# Autodesk Inventor assembly: Подъёмник
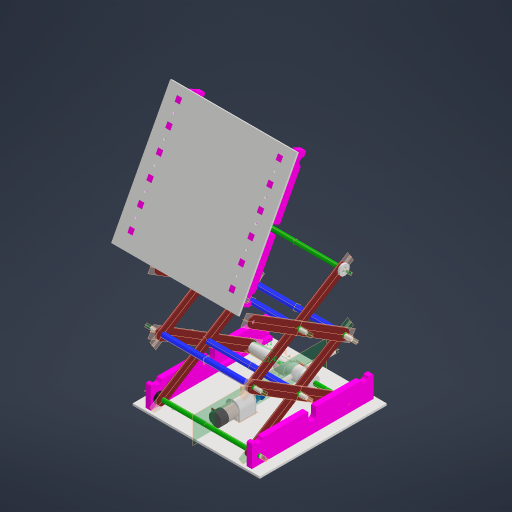
[picture p0: Inventor's stored thumbnail of the model, 512x512]
Saved by Autodesk Inventor 2023.2 (Build 272271030, 271C)
## iProperties
Created: 2025-03-18
Part Number: Подъёмник
Document SubType Name: Assembly
Designer: Коноваленко
Author: Коноваленко
## Documents named in this file (18)
- D:\!Rover\Rover\Rover_construction\Подъёмник.iam
- D:\!Rover\Rover\Rover_construction\Рельс платформы подъёмника.ipt
- D:\!Rover\Rover\Rover_construction\Рычаг платформы подъёмника.ipt
- D:\!Rover\Rover\Rover_construction\Основание подъёмника.ipt
- D:\!Rover\Rover\Rover_construction\Трубка.ipt
- D:\!Rover\Rover\Rover_construction\Рельс платформы подъёмника_MIR.ipt
- D:\!Rover\Rover\Rover_construction\Бабышка.ipt
- D:\!Rover\Rover\Rover_construction\Рельс платформы подъёмника_MIR1.ipt
- D:\!Rover\Rover\Rover_construction\Трубка основания.ipt
- D:\!Rover\Rover\Rover_construction\Подшипник.ipt
- D:\!Rover\Rover\Rover_construction\шпилька 6мм.ipt
- D:\!Rover\Rover\Rover_construction\Уголок крепления мотора.ipt
- D:\!Rover\Rover\Rover_construction\25d-metal-gearmotor-20.4-encoder.ipt
- D:\!Rover\Rover\Rover_construction\ftulka.ipt
- D:\!Rover\Rover\Rover_construction\Трапециевидный винт.ipt
- D:\!Rover\Rover\Rover_construction\Крепление ходовой гайки.ipt
- D:\!Rover\Rover\Rover_construction\THSL-300-8D õîäîâàÿ ãàéêà.ipt
- D:\!Rover\Rover\Rover_construction\Стакан для крепления ходовой гайки.ipt
## Components (60 placed, 17 different names)
1. Рельс платформы подъёмника:1 — Совмещение:63, Совмещение:64
2. Платформа подъёмника:1 — Совмещение:9, Заподлицо:8, Заподлицо:9, Заподлицо:12, Заподлицо:13, Совмещение:16, Совмещение:17, Заподлицо:14, Заподлицо:15, Совмещение:44, Заподлицо:21, Заподлицо:22
3. Рельс платформы подъёмника:4 — Совмещение:9, Заподлицо:8, Заподлицо:9, С поворотом:32, Ползун:3, Симметрия:1
4. Трубка:1 — С поворотом:82
5. Трубка:2 — С поворотом:79
6. Рельс платформы подъёмника_MIR:1 — Совмещение:65, Совмещение:66, С поворотом:86, Совмещение:81
7. Рельс платформы подъёмника_MIR1:1 — Заподлицо:12, Заподлицо:13, Совмещение:16, С поворотом:33, Ползун:4, Симметрия:1
8. Бабышка:9 — С поворотом:33, С поворотом:34
9. Бабышка:10 — С поворотом:32, С поворотом:37
10. Трубка основания:1 — С поворотом:75
11. Трубка основания:2
12. Подшипник:1 — С поворотом:70
13. Подшипник:2
14. Подшипник:3 — Ползун:3, Цилиндрический:4
15. Подшипник:4 — Ползун:4, Цилиндрический:6
16. Трубка основания:3 — С поворотом:77
17. Трубка:3 — С поворотом:72, С поворотом:77
18. Трубка:5 — С поворотом:74
19. Трубка основания:4 — С поворотом:83
20. Трубка основания:5 — С поворотом:66, С поворотом:69
21. Трубка:6 — С поворотом:54
22. Трубка:7 — С поворотом:73
23. Трубка основания:6 — Совмещение:28, Совмещение:29
24. Трубка основания:7 — С поворотом:85
25. Трубка:8 — С поворотом:53, Совмещение:28
26. Трубка:9 — Цилиндрический:2, С поворотом:66
27. шпилька 6мм:3 — С поворотом:69, С поворотом:70
28. Трубка:10 — С поворотом:84, С поворотом:85, С поворотом:86
29. Трубка основания:8 — С поворотом:80
30. Бабышка:11 — С поворотом:60
31. Бабышка:12 — С поворотом:61
32. шпилька 6мм:4 — С поворотом:71, С поворотом:72
33. шпилька 6мм:5 — С поворотом:73
34. шпилька 6мм:6 — С поворотом:74, С поворотом:75, С поворотом:76
35. шпилька 6мм:7 — С поворотом:81, С поворотом:82, С поворотом:83
36. шпилька 6мм:8 — С поворотом:84
37. шпилька 6мм:9 — С поворотом:78, С поворотом:79, С поворотом:80
38. Уголок крепления мотора:1 — Совмещение:44, Заподлицо:21, Совмещение:45, Совмещение:46, Совмещение:47, Совмещение:52
39. 25d-metal-gearmotor-20.4-encoder:1 — Совмещение:45, Совмещение:46, Совмещение:47, Совмещение:49
40. ftulka:1 — Совмещение:49, Совмещение:50, Совмещение:52, Совмещение:58
41. Трапециевидный винт:6 — Совмещение:50, Совмещение:58, Цилиндрический:1
42. Крепление ходовой гайки:1 — Совмещение:54, Совмещение:55, Совмещение:61, Совмещение:62, Совмещение:67, Совмещение:68, Совмещение:69, Совмещение:70, Совмещение:71, Совмещение:72
43. THSL-300-8D õîäîâàÿ ãàéêà:1 — Совмещение:54, Совмещение:55, Цилиндрический:1, Заподлицо:22
44. шпилька 6мм:10 — Совмещение:69, Совмещение:70, Цилиндрический:4, Цилиндрический:5, Совмещение:75
45. шпилька 6мм:11 — Совмещение:67, Совмещение:68, Цилиндрический:6, Совмещение:73
46. Трубка:11 — Совмещение:75, Совмещение:76, Совмещение:79
47. Трубка:12 — Совмещение:73, Совмещение:74, Совмещение:78
48. Трубка основания:9 — Совмещение:79, Совмещение:80
49. Трубка основания:10 — Совмещение:77, Совмещение:78
50. Стакан для крепления ходовой гайки:1 — Совмещение:61, Совмещение:62
51. Стакан для крепления ходовой гайки:2 — Совмещение:71, Совмещение:72
52. Платформа подъёмника:2 — Совмещение:63, Совмещение:64, Совмещение:65, Совмещение:66
53. Рычаг платформы подъёмника:1 — С поворотом:11, С поворотом:36, С поворотом:37
54. Рычаг платформы подъёмника:2 — С поворотом:11, С поворотом:35, С поворотом:54, С поворотом:81, Совмещение:81
55. Рычаг платформы подъёмника:3 — С поворотом:8, С поворотом:17, С поворотом:61
56. Рычаг платформы подъёмника:4 — С поворотом:8, С поворотом:15, С поворотом:71
57. Рычаг платформы подъёмника:5 — С поворотом:12, С поворотом:35, С поворотом:60, Цилиндрический:2
58. Рычаг платформы подъёмника:6 — С поворотом:12, С поворотом:36, С поворотом:53, Цилиндрический:5, Совмещение:76, Совмещение:80, С поворотом:76
59. Рычаг платформы подъёмника:7 — С поворотом:16, С поворотом:17, Совмещение:29, Совмещение:74, Совмещение:77, С поворотом:78
60. Рычаг платформы подъёмника:8 — С поворотом:15, С поворотом:16, С поворотом:34
## Relationships (87: Mate 36, RevoluteJoint 35, Flush 8, CylindricalJoint 5, TranslationJoint 2, Symmetry 1)
- Совмещение:9 [Mate]: Платформа подъёмника:1 ↔ Рельс платформы подъёмника:4
- Заподлицо:8 [Flush] (5 mm): Платформа подъёмника:1 ↔ Рельс платформы подъёмника:4
- Заподлицо:9 [Flush] (20.5 mm): Платформа подъёмника:1 ↔ Рельс платформы подъёмника:4
- С поворотом:8 [RevoluteJoint]: Рычаг платформы подъёмника:3 ↔ Рычаг платформы подъёмника:4
- С поворотом:11 [RevoluteJoint]: Рычаг платформы подъёмника:1 ↔ Рычаг платформы подъёмника:2
- С поворотом:12 [RevoluteJoint]: Рычаг платформы подъёмника:5 ↔ Рычаг платформы подъёмника:6
- С поворотом:15 [RevoluteJoint]: Рычаг платформы подъёмника:4 ↔ Рычаг платформы подъёмника:8
- С поворотом:16 [RevoluteJoint]: Рычаг платформы подъёмника:7 ↔ Рычаг платформы подъёмника:8
- С поворотом:17 [RevoluteJoint]: Рычаг платформы подъёмника:3 ↔ Рычаг платформы подъёмника:7
- Заподлицо:12 [Flush] (5 mm): Платформа подъёмника:1 ↔ Рельс платформы подъёмника_MIR1:1
- Заподлицо:13 [Flush] (20.5 mm): Платформа подъёмника:1 ↔ Рельс платформы подъёмника_MIR1:1
- Совмещение:16 [Mate]: Платформа подъёмника:1 ↔ Рельс платформы подъёмника_MIR1:1
- Совмещение:17 [Mate]: Платформа подъёмника:1
- Заподлицо:14 [Flush]: Платформа подъёмника:1
- Заподлицо:15 [Flush]: Платформа подъёмника:1
- С поворотом:32 [RevoluteJoint]: Рельс платформы подъёмника:4 ↔ Бабышка:10
- С поворотом:33 [RevoluteJoint]: Рельс платформы подъёмника_MIR1:1 ↔ Бабышка:9
- С поворотом:34 [RevoluteJoint]: Бабышка:9 ↔ Рычаг платформы подъёмника:8
- С поворотом:35 [RevoluteJoint]: Рычаг платформы подъёмника:2 ↔ Рычаг платформы подъёмника:5
- С поворотом:36 [RevoluteJoint]: Рычаг платформы подъёмника:1 ↔ Рычаг платформы подъёмника:6
- С поворотом:37 [RevoluteJoint]: Бабышка:10 ↔ Рычаг платформы подъёмника:1
- Ползун:3 [TranslationJoint]: Рельс платформы подъёмника:4 ↔ Подшипник:3
- Ползун:4 [TranslationJoint]: Рельс платформы подъёмника_MIR1:1 ↔ Подшипник:4
- С поворотом:53 [RevoluteJoint] (-0.5 mm): Трубка:8 ↔ Рычаг платформы подъёмника:6
- С поворотом:54 [RevoluteJoint] (-11.5 mm): Трубка:6 ↔ Рычаг платформы подъёмника:2
- Совмещение:28 [Mate]: Трубка основания:6 ↔ Трубка:8
- Совмещение:29 [Mate] (0.5 mm): Трубка основания:6 ↔ Рычаг платформы подъёмника:7
- С поворотом:60 [RevoluteJoint] (-4.5 mm): Бабышка:11 ↔ Рычаг платформы подъёмника:5
- С поворотом:61 [RevoluteJoint] (-0.5 mm): Бабышка:12 ↔ Рычаг платформы подъёмника:3
- Совмещение:44 [Mate]: Платформа подъёмника:1 ↔ Уголок крепления мотора:1
- Заподлицо:21 [Flush]: Платформа подъёмника:1 ↔ Уголок крепления мотора:1
- Совмещение:45 [Mate]: Уголок крепления мотора:1 ↔ 25d-metal-gearmotor-20.4-encoder:1
- Совмещение:46 [Mate]: Уголок крепления мотора:1 ↔ 25d-metal-gearmotor-20.4-encoder:1
- Совмещение:47 [Mate]: Уголок крепления мотора:1 ↔ 25d-metal-gearmotor-20.4-encoder:1
- Совмещение:49 [Mate]: 25d-metal-gearmotor-20.4-encoder:1 ↔ ftulka:1
- Совмещение:50 [Mate]: ftulka:1 ↔ Трапециевидный винт:6
- Совмещение:52 [Mate] (2 mm): Уголок крепления мотора:1 ↔ ftulka:1
- Совмещение:54 [Mate]: Крепление ходовой гайки:1 ↔ THSL-300-8D õîäîâàÿ ãàéêà:1
- Совмещение:55 [Mate]: Крепление ходовой гайки:1 ↔ THSL-300-8D õîäîâàÿ ãàéêà:1
- Совмещение:58 [Mate] (-10 mm): ftulka:1 ↔ Трапециевидный винт:6
- Цилиндрический:1 [CylindricalJoint]: Трапециевидный винт:6 ↔ THSL-300-8D õîäîâàÿ ãàéêà:1
- Заподлицо:22 [Flush]: Платформа подъёмника:1 ↔ THSL-300-8D õîäîâàÿ ãàéêà:1
- Совмещение:61 [Mate]: Крепление ходовой гайки:1 ↔ Стакан для крепления ходовой гайки:1
- Совмещение:62 [Mate]: Крепление ходовой гайки:1 ↔ Стакан для крепления ходовой гайки:1
- Совмещение:63 [Mate]: Рельс платформы подъёмника:1 ↔ Платформа подъёмника:2
- Совмещение:64 [Mate]: Рельс платформы подъёмника:1 ↔ Платформа подъёмника:2
- Совмещение:65 [Mate]: Рельс платформы подъёмника_MIR:1 ↔ Платформа подъёмника:2
- Совмещение:66 [Mate]: Рельс платформы подъёмника_MIR:1 ↔ Платформа подъёмника:2
- Цилиндрический:2 [CylindricalJoint]: Трубка:9 ↔ Рычаг платформы подъёмника:5
- Совмещение:67 [Mate]: Крепление ходовой гайки:1 ↔ шпилька 6мм:11
- Совмещение:68 [Mate]: Крепление ходовой гайки:1 ↔ шпилька 6мм:11
- Совмещение:69 [Mate]: Крепление ходовой гайки:1 ↔ шпилька 6мм:10
- Совмещение:70 [Mate]: Крепление ходовой гайки:1 ↔ шпилька 6мм:10
- Совмещение:71 [Mate]: Крепление ходовой гайки:1 ↔ Стакан для крепления ходовой гайки:2
- Совмещение:72 [Mate]: Крепление ходовой гайки:1 ↔ Стакан для крепления ходовой гайки:2
- Цилиндрический:4 [CylindricalJoint]: Подшипник:3 ↔ шпилька 6мм:10
- Цилиндрический:5 [CylindricalJoint]: шпилька 6мм:10 ↔ Рычаг платформы подъёмника:6
- Цилиндрический:6 [CylindricalJoint]: Подшипник:4 ↔ шпилька 6мм:11
- С поворотом:66 [RevoluteJoint]: Трубка основания:5 ↔ Трубка:9
- С поворотом:69 [RevoluteJoint]: Трубка основания:5 ↔ шпилька 6мм:3
- С поворотом:70 [RevoluteJoint] (0.5 mm): Подшипник:1 ↔ шпилька 6мм:3
- Совмещение:73 [Mate]: шпилька 6мм:11 ↔ Трубка:12
- Совмещение:74 [Mate] (0.5 mm): Трубка:12 ↔ Рычаг платформы подъёмника:7
- Совмещение:75 [Mate]: шпилька 6мм:10 ↔ Трубка:11
- Совмещение:76 [Mate] (0.5 mm): Трубка:11 ↔ Рычаг платформы подъёмника:6
- Совмещение:77 [Mate] (0.5 mm): Трубка основания:10 ↔ Рычаг платформы подъёмника:7
- Совмещение:78 [Mate]: Трубка:12 ↔ Трубка основания:10
- Совмещение:79 [Mate]: Трубка:11 ↔ Трубка основания:9
- Совмещение:80 [Mate] (0.5 mm): Трубка основания:9 ↔ Рычаг платформы подъёмника:6
- С поворотом:71 [RevoluteJoint] (-15 mm): шпилька 6мм:4 ↔ Рычаг платформы подъёмника:4
- С поворотом:72 [RevoluteJoint]: Трубка:3 ↔ шпилька 6мм:4
- С поворотом:73 [RevoluteJoint]: Трубка:7 ↔ шпилька 6мм:5
- С поворотом:74 [RevoluteJoint]: Трубка:5 ↔ шпилька 6мм:6
- С поворотом:75 [RevoluteJoint]: Трубка основания:1 ↔ шпилька 6мм:6
- С поворотом:76 [RevoluteJoint] (-15 mm): шпилька 6мм:6 ↔ Рычаг платформы подъёмника:6
- С поворотом:77 [RevoluteJoint]: Трубка основания:3 ↔ Трубка:3
- С поворотом:78 [RevoluteJoint] (-15 mm): шпилька 6мм:9 ↔ Рычаг платформы подъёмника:7
- С поворотом:79 [RevoluteJoint]: Трубка:2 ↔ шпилька 6мм:9
- С поворотом:80 [RevoluteJoint]: Трубка основания:8 ↔ шпилька 6мм:9
- С поворотом:81 [RevoluteJoint] (-15 mm): шпилька 6мм:7 ↔ Рычаг платформы подъёмника:2
- С поворотом:82 [RevoluteJoint]: Трубка:1 ↔ шпилька 6мм:7
- С поворотом:83 [RevoluteJoint]: Трубка основания:4 ↔ шпилька 6мм:7
- С поворотом:84 [RevoluteJoint]: Трубка:10 ↔ шпилька 6мм:8
- С поворотом:85 [RevoluteJoint]: Трубка основания:7 ↔ Трубка:10
- С поворотом:86 [RevoluteJoint] (2 mm): Рельс платформы подъёмника_MIR:1 ↔ Трубка:10
- Совмещение:81 [Mate] (0.5 mm): Рельс платформы подъёмника_MIR:1 ↔ Рычаг платформы подъёмника:2
- Симметрия:1 [Symmetry]: Рельс платформы подъёмника:4 ↔ Рельс платформы подъёмника_MIR1:1
